# Autodesk Inventor assembly: Shipping goods generic subassembly
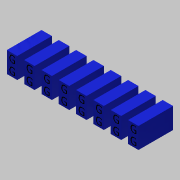
[picture p0: Inventor's stored thumbnail of the model, 180x180]
Saved by Autodesk Inventor 2015 (Build 190159000, 159)
## iProperties
Created: 2015-03-08
Part Number: Shipping goods generic subassembly
Document SubType Name: Assembly
Designer: Vukica
Author: Vukica
## Documents named in this file (2)
- D:\Dropbox\Dropbox\Service\IEEE\!Final Rules\2016Hardware_Court_v8-aug12\Shipping goods generic subassembly.iam
- D:\Dropbox\Dropbox\Service\IEEE\!Final Rules\2016Hardware_Court_v8-aug12\Container 2 2 5 generic.ipt
## Components (16 placed, 1 different names)
1. Container 2 2 5 generic:1 — Mate:1, Flush:1, Flush:5, Mate:9, Flush:35
2. Container 2 2 5 generic:2 — Mate:1, Mate:2, Flush:1, Flush:2, Flush:5, Flush:6
3. Container 2 2 5 generic:3 — Mate:2, Flush:2, Flush:6
4. Container 2 2 5 generic:6 — Mate:9, Mate:13, Flush:24, Flush:25, Flush:26, Flush:35
5. Container 2 2 5 generic:7
6. Container 2 2 5 generic:8 — Mate:20, Flush:38, Flush:39
7. Container 2 2 5 generic:11 — Flush:23, Mate:14, Flush:27, Flush:28
8. Container 2 2 5 generic:12 — Flush:25
9. Container 2 2 5 generic:13 — Flush:23, Flush:31, Flush:32
10. Container 2 2 5 generic:14 — Mate:13, Flush:24, Flush:26
11. Container 2 2 5 generic:15 — Mate:14, Flush:27, Flush:28, Mate:15, Flush:29, Flush:30, Mate:16
12. Container 2 2 5 generic:16 — Mate:15, Flush:29, Flush:30, Mate:17, Flush:33
13. Container 2 2 5 generic:17 — Mate:16, Flush:31, Flush:32, Flush:34, Mate:18
14. Container 2 2 5 generic:18 — Mate:17, Flush:33, Flush:34, Mate:18
15. Container 2 2 5 generic:19 — Mate:19, Flush:36, Flush:37, Mate:20, Flush:38, Flush:39
16. Container 2 2 5 generic:20 — Mate:19, Flush:36, Flush:37
## Relationships (45: Flush 29, Mate 16)
- Mate:1 (25.4 mm): Container 2 2 5 generic:1 ↔ Container 2 2 5 generic:2
- Mate:2 (25.4 mm): Container 2 2 5 generic:2 ↔ Container 2 2 5 generic:3
- Flush:1: Container 2 2 5 generic:1 ↔ Container 2 2 5 generic:2
- Flush:2: Container 2 2 5 generic:2 ↔ Container 2 2 5 generic:3
- Flush:5: Container 2 2 5 generic:1 ↔ Container 2 2 5 generic:2
- Flush:6: Container 2 2 5 generic:2 ↔ Container 2 2 5 generic:3
- [Mate] (25.4 mm): Container 2 2 5 generic:6 ↔ Container 2 2 5 generic:7
- [Mate] (25.4 mm): Container 2 2 5 generic:7 ↔ Container 2 2 5 generic:8
- [Flush]: Container 2 2 5 generic:6 ↔ Container 2 2 5 generic:7
- [Flush]: Container 2 2 5 generic:7 ↔ Container 2 2 5 generic:8
- [Flush]: Container 2 2 5 generic:6 ↔ Container 2 2 5 generic:7
- [Flush]: Container 2 2 5 generic:7 ↔ Container 2 2 5 generic:8
- Mate:9: Container 2 2 5 generic:1 ↔ Container 2 2 5 generic:6
- [Mate] (25.4 mm): Container 2 2 5 generic:11 ↔ Container 2 2 5 generic:12
- [Flush]: Container 2 2 5 generic:11 ↔ Container 2 2 5 generic:12
- [Flush]: Container 2 2 5 generic:11 ↔ Container 2 2 5 generic:12
- [Mate] (25.4 mm): Container 2 2 5 generic:13 ↔ Container 2 2 5 generic:14
- [Flush]: Container 2 2 5 generic:13 ↔ Container 2 2 5 generic:14
- [Flush]: Container 2 2 5 generic:13 ↔ Container 2 2 5 generic:14
- [Mate]: Container 2 2 5 generic:11 ↔ Container 2 2 5 generic:13
- Mate:13 (25.4 mm): Container 2 2 5 generic:6 ↔ Container 2 2 5 generic:14
- Flush:23: Container 2 2 5 generic:11 ↔ Container 2 2 5 generic:13
- Flush:24: Container 2 2 5 generic:6 ↔ Container 2 2 5 generic:14
- Flush:25: Container 2 2 5 generic:6 ↔ Container 2 2 5 generic:12
- Flush:26: Container 2 2 5 generic:6 ↔ Container 2 2 5 generic:14
- Mate:14 (25.4 mm): Container 2 2 5 generic:11 ↔ Container 2 2 5 generic:15
- Flush:27: Container 2 2 5 generic:11 ↔ Container 2 2 5 generic:15
- Flush:28: Container 2 2 5 generic:11 ↔ Container 2 2 5 generic:15
- Mate:15 (25.4 mm): Container 2 2 5 generic:15 ↔ Container 2 2 5 generic:16
- Flush:29: Container 2 2 5 generic:15 ↔ Container 2 2 5 generic:16
- Flush:30: Container 2 2 5 generic:15 ↔ Container 2 2 5 generic:16
- Mate:16: Container 2 2 5 generic:15 ↔ Container 2 2 5 generic:17
- Flush:31: Container 2 2 5 generic:13 ↔ Container 2 2 5 generic:17
- Flush:32: Container 2 2 5 generic:13 ↔ Container 2 2 5 generic:17
- Mate:17: Container 2 2 5 generic:16 ↔ Container 2 2 5 generic:18
- Flush:33: Container 2 2 5 generic:16 ↔ Container 2 2 5 generic:18
- Flush:34: Container 2 2 5 generic:17 ↔ Container 2 2 5 generic:18
- Mate:18 (25.4 mm): Container 2 2 5 generic:17 ↔ Container 2 2 5 generic:18
- Flush:35: Container 2 2 5 generic:1 ↔ Container 2 2 5 generic:6
- Mate:19: Container 2 2 5 generic:19 ↔ Container 2 2 5 generic:20
- Flush:36: Container 2 2 5 generic:19 ↔ Container 2 2 5 generic:20
- Flush:37: Container 2 2 5 generic:19 ↔ Container 2 2 5 generic:20
- Mate:20 (25.4 mm): Container 2 2 5 generic:8 ↔ Container 2 2 5 generic:19
- Flush:38: Container 2 2 5 generic:8 ↔ Container 2 2 5 generic:19
- Flush:39: Container 2 2 5 generic:8 ↔ Container 2 2 5 generic:19
## Named parameters: d12_d0 = 25.4 mm, d13_d1 = 25.4 mm, d16_d4 = 0 mm, d17_d5 = 0 mm, d20_d8 = 0 mm, d21_d9 = 0 mm, d27_d0 = 25.4 mm, d28_d4 = 0 mm, d29_d8 = 0 mm, d30_d12_d0 = 25.4 mm, d31_d16_d4 = 0 mm, d32_d20_d8 = 0 mm, d33_d24 = 0 mm
